# Autodesk Inventor assembly: 32blit
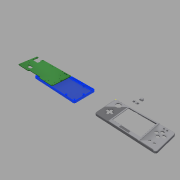
[picture p0: Inventor's stored thumbnail of the model, 180x180]
Saved by Autodesk Inventor 2019 (Build 230136000, 136)
## iProperties
Created: 2019-09-09
Part Number: 32blit
Document SubType Name: Assembly
Designer: jon
Author: jon
## Documents named in this file (6)
- C:\Users\jon\Documents\GitHub\X\mechanical\case-new\32blit.iam
- C:\Users\jon\Documents\GitHub\X\mechanical\case-new\pcb.ipt
- C:\Users\jon\Documents\GitHub\X\mechanical\case-new\base.ipt
- C:\Users\jon\Documents\GitHub\X\mechanical\case-new\top.ipt
- C:\Users\jon\Documents\GitHub\X\mechanical\case-new\action-button.ipt
- C:\Users\jon\Documents\GitHub\X\mechanical\case-new\system-buttons.ipt
## Components (5 placed, 5 different names)
1. pcb:1 — Flush:1, Mate:1, Mate:2, Flush:4
2. base:1 — Flush:1, Mate:1, Flush:2, Flush:3
3. top:1 — Mate:2, Flush:2, Flush:3, Flush:4, Flush:5, Flush:6
4. action-button:1 — Flush:5
5. system-buttons:1 — Flush:6
## Relationships (8: Flush 6, Mate 2)
- Flush:1 (2 mm): pcb:1 ↔ base:1
- Mate:1: pcb:1 ↔ base:1
- Mate:2: pcb:1 ↔ top:1
- Flush:2: base:1 ↔ top:1
- Flush:3: base:1 ↔ top:1
- Flush:4 (2 mm): pcb:1 ↔ top:1
- Flush:5 (-0.5 mm): top:1 ↔ action-button:1
- Flush:6: top:1 ↔ system-buttons:1
